# Autodesk Inventor assembly: Controlpanel
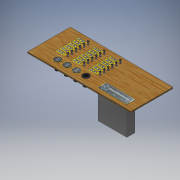
[picture p0: Inventor's stored thumbnail of the model, 180x180]
Saved by Autodesk Inventor 2019.2 (Build 232265000, 265)
## iProperties
Created: 2020-05-18
Part Number: Controlpanel
Document SubType Name: Assembly
Designer: Johansson
Author: Johansson
## Documents named in this file (9)
- D:\Dropbox\Dokument\Projekt\Elita\Electrical system\Highside-Powerdistribution\hardware\control-panel\Controlpanel.iam
- D:\Dropbox\Dokument\Projekt\Elita\Electrical system\Highside-Powerdistribution\hardware\control-panel\wooden-panel.ipt
- D:\Dropbox\Dokument\Projekt\Elita\Electrical system\Highside-Powerdistribution\hardware\control-panel\label.ipt
- D:\Dropbox\Dokument\Inventor\Content Center Files\R2019\en-US\CNS 9671\CNS 9671 - M2,3 x 5.ipt
- D:\Dropbox\Dokument\Projekt\Elita\Electrical system\Highside-Powerdistribution\hardware\control-panel\stereo.ipt
- D:\Dropbox\Dokument\Projekt\Elita\Electrical system\Highside-Powerdistribution\hardware\control-panel\usb_outlet.ipt
- D:\Dropbox\Dokument\Projekt\Elita\Electrical system\Highside-Powerdistribution\hardware\control-panel\12v_outlet.ipt
- D:\Dropbox\Dokument\Projekt\Elita\Electrical system\Highside-Powerdistribution\hardware\control-panel\dragswitch.ipt
- D:\Dropbox\Dokument\Projekt\Elita\Electrical system\Highside-Powerdistribution\hardware\control-panel\parameters.xlsx
## Components (78 placed, 7 different names)
1. wooden-panel:1 — Mate:2, Mate:3, Mate:4, Mate:5, Mate:6, Mate:7, Mate:8, Mate:9, Mate:10, Mate:11
2. stereo:1 — Mate:3, Mate:4, Mate:5
3. 12v_outlet:1 — Mate:8, Mate:9
4. label:5 — Mate:2, Insert:3, Insert:4
5. CNS 9671 M2,3 x 5:9 — Insert:3
6. CNS 9671 M2,3 x 5:10 — Insert:4
7. label:6
8. CNS 9671 M2,3 x 5:11
9. CNS 9671 M2,3 x 5:12
10. label:7
11. CNS 9671 M2,3 x 5:13
12. CNS 9671 M2,3 x 5:14
13. label:8
14. CNS 9671 M2,3 x 5:15
15. CNS 9671 M2,3 x 5:16
16. label:9
17. CNS 9671 M2,3 x 5:17
18. CNS 9671 M2,3 x 5:18
19. label:10
20. CNS 9671 M2,3 x 5:19
21. CNS 9671 M2,3 x 5:20
22. label:11
23. CNS 9671 M2,3 x 5:21
24. CNS 9671 M2,3 x 5:22
25. label:12
26. CNS 9671 M2,3 x 5:23
27. CNS 9671 M2,3 x 5:24
28. label:13
29. CNS 9671 M2,3 x 5:25
30. CNS 9671 M2,3 x 5:26
31. label:14
32. CNS 9671 M2,3 x 5:27
33. CNS 9671 M2,3 x 5:28
34. label:15
35. CNS 9671 M2,3 x 5:29
36. CNS 9671 M2,3 x 5:30
37. label:16
38. CNS 9671 M2,3 x 5:31
39. CNS 9671 M2,3 x 5:32
40. label:17
41. CNS 9671 M2,3 x 5:33
42. CNS 9671 M2,3 x 5:34
43. label:18
44. CNS 9671 M2,3 x 5:35
45. CNS 9671 M2,3 x 5:36
46. label:19
47. CNS 9671 M2,3 x 5:37
48. CNS 9671 M2,3 x 5:38
49. label:20
50. CNS 9671 M2,3 x 5:39
51. CNS 9671 M2,3 x 5:40
52. label:21
53. CNS 9671 M2,3 x 5:41
54. CNS 9671 M2,3 x 5:42
55. label:22
56. CNS 9671 M2,3 x 5:43
57. CNS 9671 M2,3 x 5:44
58. usb_outlet:1 — Mate:6, Mate:7
59. usb_outlet:2
60. usb_outlet:3
61. dragswitch:1 — Mate:10, Mate:11
62. dragswitch:2
63. dragswitch:3
64. dragswitch:4
65. dragswitch:5
66. dragswitch:6
67. dragswitch:7
68. dragswitch:8
69. dragswitch:9
70. dragswitch:10
71. dragswitch:11
72. dragswitch:12
73. dragswitch:13
74. dragswitch:14
75. dragswitch:15
76. dragswitch:16
77. dragswitch:17
78. dragswitch:18
## Component patterns: (18 elements, first: label:5 + CNS 9671 M2,3 x 5:9 + CNS 9671 M2,3 x 5:10), (3 elements, first: usb_outlet:1), (18 elements, first: dragswitch:1)
## Relationships (12: Mate 10, Insert 2)
- Mate:2: wooden-panel:1 ↔ label:5
- Insert:3: label:5 ↔ CNS 9671 M2,3 x 5:9
- Insert:4: label:5 ↔ CNS 9671 M2,3 x 5:10
- Mate:3: wooden-panel:1 ↔ stereo:1
- Mate:4: wooden-panel:1 ↔ stereo:1
- Mate:5: wooden-panel:1 ↔ stereo:1
- Mate:6: wooden-panel:1 ↔ usb_outlet:1
- Mate:7: wooden-panel:1 ↔ usb_outlet:1
- Mate:8: wooden-panel:1 ↔ 12v_outlet:1
- Mate:9: wooden-panel:1 ↔ 12v_outlet:1
- Mate:10: wooden-panel:1 ↔ dragswitch:1
- Mate:11: wooden-panel:1 ↔ dragswitch:1
## Named parameters: wl_panel = 265 mm, wr_panel = 260 mm, l_panel = 640 mm, t_panel = 8 mm, r_button = 8 mm, l_stereo = 178 mm, w_stereo = 50 mm, d_stereo = 177 mm, w_label = 15 mm, l_label = 50 mm, n_navlights = 4, r_labelscrew = 2.5 mm, ro_labelscrew = 5 mm, l_buttontobutton = 25 mm, n_interior = 6, r_usboutlet = 29 mm, n_usboutlets = 4, l_fastener_button = 19 mm
